# Autodesk Inventor assembly: 900-50-PROFILES-ANGLE-CONN-20x20-01-N6_N8
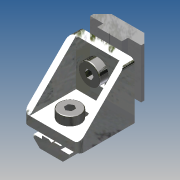
[picture p0: Inventor's stored thumbnail of the model, 180x180]
Saved by Autodesk Inventor 2018.2 (Build 222227000, 227)
## iProperties
Manager: feesmrt
Company: FRANCOR
Part Number: 900-50-PROFILES-ANGLE-CONN-20x20-01-N6_N8
Project: Rescue Robot
Cost Center: -
Material: Generisch
Document SubType Name: Assembly
Designer: feesmrt
Engineer: feesmrt
Authority: feesmrt
Description: Profile Connector ASM N6 N8
Stock Number: 900-50-PROFILES-ANGLE-CONN-20x20-01-N6_N8
Subject: Rescue Robot
Author: feesmrt
Revision Number: 1
Title: Profile Connector ASM N6 N8
## Documents named in this file (6)
- D:\Programmierung\FRANC0R\CAD\02-Rocker-Bogie-Robot\900-COMPONENTS\900-50-PROFILES\900-50-PROFILES-ANGLE-CONN-20x20-01-N6_N8.iam
- D:\Programmierung\FRANC0R\CAD\02-Rocker-Bogie-Robot\900-COMPONENTS\900-50-PROFILES\900-50-PROFILES-ANGLE-CONN-20x20.ipt
- D:\Programmierung\FRANC0R\CAD\02-Rocker-Bogie-Robot\900-COMPONENTS\900-40-SCREWS\900-40-SCREWS-DIN7984_M4x8.ipt
- D:\Programmierung\FRANC0R\CAD\02-Rocker-Bogie-Robot\900-COMPONENTS\900-50-PROFILES\900-50-PROFILES-CONN-N6xM4.ipt
- D:\Programmierung\FRANC0R\CAD\02-Rocker-Bogie-Robot\900-COMPONENTS\900-50-PROFILES\900-50-PROFILES-CONN-N8xM4.ipt
- D:\Programmierung\FRANC0R\CAD\02-Rocker-Bogie-Robot\900-COMPONENTS\900-40-SCREWS\900-40-SCREWS-DIN7984_M4x10.ipt
## Components (5 placed, 5 different names)
1. 900-50-PROFILES-ANGLE-CONN-20x20:1 — Passend:1, Passend:4, Passend:9, Passend:12, Passend:13, Passend:16
2. 900-40-SCREWS-DIN7984_M4x8:1 — Passend:1, Passend:4, Passend:6, Passend:8
3. 900-50-PROFILES-CONN-N6xM4:1 — Passend:8, Passend:9, Passend:11
4. 900-40-SCREWS-DIN7984_M4x10:1 — Passend:12, Passend:13, Passend:14, Passend:15
5. 900-50-PROFILES-CONN-N8xM4:1 — Passend:15, Passend:16, Passend:17
## Relationships (12: Mate 12)
- Passend:1 [Mate]: 900-50-PROFILES-ANGLE-CONN-20x20:1 ↔ 900-40-SCREWS-DIN7984_M4x8:1
- Passend:4 [Mate] (-12 mm): 900-50-PROFILES-ANGLE-CONN-20x20:1 ↔ 900-40-SCREWS-DIN7984_M4x8:1
- Passend:6 [Mate]: 900-40-SCREWS-DIN7984_M4x8:1
- Passend:8 [Mate]: 900-40-SCREWS-DIN7984_M4x8:1 ↔ 900-50-PROFILES-CONN-N6xM4:1
- Passend:9 [Mate] (1.5 mm): 900-50-PROFILES-ANGLE-CONN-20x20:1 ↔ 900-50-PROFILES-CONN-N6xM4:1
- Passend:11 [Mate]: 900-50-PROFILES-CONN-N6xM4:1
- Passend:12 [Mate]: 900-50-PROFILES-ANGLE-CONN-20x20:1 ↔ 900-40-SCREWS-DIN7984_M4x10:1
- Passend:13 [Mate] (-12 mm): 900-50-PROFILES-ANGLE-CONN-20x20:1 ↔ 900-40-SCREWS-DIN7984_M4x10:1
- Passend:14 [Mate]: 900-40-SCREWS-DIN7984_M4x10:1
- Passend:15 [Mate]: 900-40-SCREWS-DIN7984_M4x10:1 ↔ 900-50-PROFILES-CONN-N8xM4:1
- Passend:16 [Mate] (2.8 mm): 900-50-PROFILES-ANGLE-CONN-20x20:1 ↔ 900-50-PROFILES-CONN-N8xM4:1
- Passend:17 [Mate]: 900-50-PROFILES-CONN-N8xM4:1
